# Autodesk Inventor assembly: SCST8-15
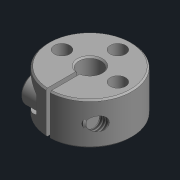
[picture p0: Inventor's stored thumbnail of the model, 180x180]
Saved by Autodesk Inventor 2022 (Build 260153000, 153)
## iProperties
Part Number: SCST8-15
Catalog Web Link: www.cadenas.de
Description: SCST, PSCST, SSCST, SCSTR, PSCSTR, SSCSTR-Shaft Collars - 3 Holes/3 Taps
Vendor: MISUMI
Document SubType Name: Assembly
Designer: partserver
Manufacturer: MISUMI
Mass: 8.24389 g
Surface Area: 49.0146 cm^2
Volume: 8.24389 cm^3
Density: 1 g/cm^3
Category: PARTsolutions
Company: MISUMI
PSOL_IDENT_0: {$CADENAS_DATA\23d-libs\misumi\metric\03_set_collars\scst_asmtab.prj},219 {VTYP=3D},{STYP=ASSTAB},{N
PSOL_IDENT_1: B=SCST8-15},{LINA=SCST8-15},{NN=SCST, PSCST, SSCST, SCSTR, PSCSTR, SSCSTR},{DATE=30.06.2021 12:52:05
PSOL_IDENT_2: },{GEOMDATE=30.10.2015 01:45:58},{VERSION=},{LINEID=50},{WBVAR=TS,MAT,ST,BS},{WBNUMERIC=BS}  {NB=SCS
PSOL_IDENT_3: T8-15},{LINA=SCST8-15},{KT=DUMMY},{PN=SCST8-15},{TYPE=SCST},{TS=3H},{TSALG= '3H' , '3-Hole' , '3T' ,
PSOL_IDENT_4: '3-Tapped' },{MAT=S45C},{ST=BO},{STALG= 'BO' , 'Black Oxide' , 'ENP' , 'Electroless Nickel Plating'
PSOL_IDENT_5: },{AC=Hex Socket Head Cap Screw 1 pc.},{ACMAT=4137 Alloy Steel},{D=8},{BS=15},{BALG= 8 , 10 , 15 },
PSOL_IDENT_6: {D1=30},{M=M6},{M3D=6},{DD=6.6},{R=6.00},{W=1.5},{X=9.0},{Y=5},{P=20},{C=0.5},{S=5.5},{M1=-},{M13D=0
PSOL_IDENT_7: },{L=15},{PPATH=scst/scst_templ.prj}
NB: SCST8-15
NN: SCST, PSCST, SSCST, SCSTR, PSCSTR, SSCSTR
NT: Shaft Collars - 3 Holes/3 Taps
NBSYN: $PN.
LINA: SCST8-15
CATALOG: Misumi
PN: SCST8-15
TS: 3-Hole
MAT: 1045 Carbon Steel
ST: Black Oxide
AC: Hex Socket Head Cap Screw 1 pc.
ACMAT: 4137 Alloy Steel
D: 8
BS: 15
D1: 30
M: M6
DD: 6.6
R: 6
W: 1.5
X: 9
Y: 5
P: 20
C: 0.5
S: 5.5
M1: -
SUPPLIER: MISUMI
ARTICLENO: SCST8-15
BOMINFO: SCST8-15
CREATOR: CADENAS GmbH
Title: SCST8-15
Author: Cadenas PARTsolutions
Comments: Shaft Collars - 3 Holes/3 Taps
## Documents named in this file (3)
- C:\Users\yuta0\Documents\GitHub\catchrobo_hardware\assy-shooter\SCST8-15.iam
- C:\Users\yuta0\Documents\GitHub\catchrobo_hardware\assy-shooter\SCST8-15b.ipt
- C:\Users\yuta0\Documents\GitHub\catchrobo_hardware\assy-shooter\BOLT6-15.ipt
## Components (2 placed, 2 different names)
1. SCST8-15b:1 — to_bolt_XY@1 <-> to_cp_XY@2, to_bolt_Z@1 <-> to_cp_Z@2, to_bolt_YZ@1 <-> to_cp_YZ@2
2. BOLT6-15:1 — to_bolt_XY@1 <-> to_cp_XY@2, to_bolt_Z@1 <-> to_cp_Z@2, to_bolt_YZ@1 <-> to_cp_YZ@2
## Relationships (3: Mate 2, Angle 1)
- to_bolt_XY@1 <-> to_cp_XY@2 [Mate]: SCST8-15b:1 ↔ BOLT6-15:1
- to_bolt_Z@1 <-> to_cp_Z@2 [Mate]: SCST8-15b:1 ↔ BOLT6-15:1
- to_bolt_YZ@1 <-> to_cp_YZ@2 [Angle] (0 deg): SCST8-15b:1 ↔ BOLT6-15:1
